# Autodesk Inventor assembly: structure_front
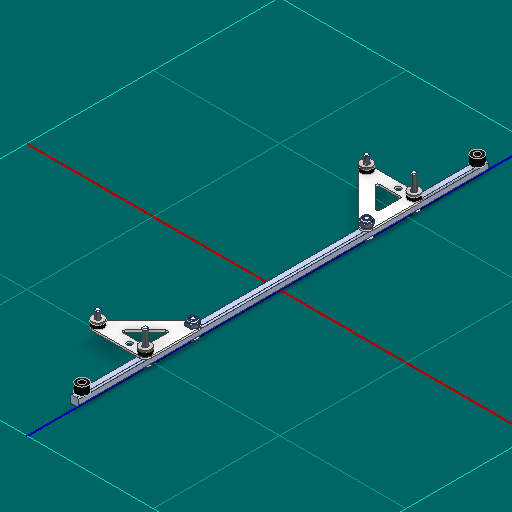
[picture p0: Inventor's stored thumbnail of the model, 512x512]
Saved by Autodesk Inventor 2025 (Build 290162000, 162)
## iProperties
Created: 2024-08-21
Part Number: structure_front
Document SubType Name: Assembly
Designer: averey
Author: averey
## Documents named in this file (12)
- C:\Users\avere\vex_robotics_high_stakes\hardware\cad\bots\ENIGMA\chassis\drivetrain\structure\structure_front.iam
- C:\Users\avere\vex_robotics_high_stakes\hardware\cad\bots\ENIGMA\chassis\drivetrain\structure\custom_parts\hs_crossbrace.ipt
- C:\Users\avere\vex_robotics_high_stakes\hardware\cad\bots\ENIGMA\chassis\drivetrain\structure\custom_parts\right_angle_gusset.ipt
- C:\Users\avere\vex_robotics_high_stakes\hardware\cad\VEX-CAD-Inventor\Structure\Hardware\Screw Steel - Star.ipt
- C:\Users\avere\vex_robotics_high_stakes\hardware\cad\VEX-CAD-Inventor\Motion\Spacers\Spacer Nylon .375 OD\NSpacer .375 OD x .125.ipt
- C:\Users\avere\vex_robotics_high_stakes\hardware\cad\VEX-CAD-Inventor\Motion\Spacers\Spacer Nylon .375 OD.ipt
- C:\Users\avere\vex_robotics_high_stakes\hardware\cad\VEX-CAD-Inventor\Motion\Spacers\Washer Steel\SWasher .375 OD x .062500.ipt
- C:\Users\avere\vex_robotics_high_stakes\hardware\cad\VEX-CAD-Inventor\Motion\Spacers\Washer Steel.ipt
- C:\Users\avere\vex_robotics_high_stakes\hardware\cad\VEX-CAD-Inventor\Motion\Spacers\Spacer Nylon .375 OD\NSpacer .375 OD x .250.ipt
- C:\Users\avere\vex_robotics_high_stakes\hardware\cad\VEX-CAD-Inventor\Structure\Hardware\Screw Steel - Star\SScrew Star Smooth .500.ipt
- C:\Users\avere\vex_robotics_high_stakes\hardware\cad\VEX-CAD-Inventor\Structure\Hardware\Nut Thin Nylock.ipt
- C:\Users\avere\vex_robotics_high_stakes\hardware\cad\VEX-CAD-Inventor\Structure\Hardware\Screw Steel - Star\SScrew Star Smooth 1.000.ipt
## Components (21 placed, 8 different names)
1. hs_crossbrace:1 — Mate:1, Insert:1, Mate:2, Insert:2, Mate:3, Insert:15, Insert:16, Insert:23, Insert:24, Insert:27, Insert:28
2. right_angle_gusset:1 — Insert:1, Mate:2, Insert:14, Insert:18, Insert:21, Insert:26
3. right_angle_gusset:2 — Insert:2, Mate:3, Insert:10, Insert:20, Insert:22, Insert:25
4. NSpacer .375 OD x .125:3 — Insert:10
5. SWasher .375 OD x .062500:2
6. NSpacer .375 OD x .125:5 — Insert:14
7. SWasher .375 OD x .062500:4
8. NSpacer .375 OD x .250:6 — Insert:15
9. NSpacer .375 OD x .250:7 — Insert:16
10. NSpacer .375 OD x .125:8 — Insert:18
11. SWasher .375 OD x .062500:5
12. NSpacer .375 OD x .125:9 — Insert:20
13. SWasher .375 OD x .062500:6
14. SScrew Star Smooth .500:6 — Insert:21
15. SScrew Star Smooth .500:7 — Insert:22
16. SScrew Star Smooth .500:8 — Insert:23
17. SScrew Star Smooth .500:9 — Insert:24
18. Nut Thin Nylock:1 — Insert:25
19. Nut Thin Nylock:2 — Insert:26
20. SScrew Star Smooth 1.000:10 — Insert:27
21. SScrew Star Smooth 1.000:11 — Insert:28
## Relationships (23: Insert 20, Mate 3)
- Mate:1 (-165.1 mm): hs_crossbrace:1
- Insert:1: hs_crossbrace:1 ↔ right_angle_gusset:1
- Mate:2: hs_crossbrace:1 ↔ right_angle_gusset:1
- Insert:2: hs_crossbrace:1 ↔ right_angle_gusset:2
- Mate:3: hs_crossbrace:1 ↔ right_angle_gusset:2
- [Insert]: NSpacer .375 OD x .125:3 ↔ SWasher .375 OD x .062500:2
- Insert:10: right_angle_gusset:2 ↔ NSpacer .375 OD x .125:3
- [Insert]: NSpacer .375 OD x .125:5 ↔ SWasher .375 OD x .062500:4
- Insert:14: right_angle_gusset:1 ↔ NSpacer .375 OD x .125:5
- Insert:15: hs_crossbrace:1 ↔ NSpacer .375 OD x .250:6
- Insert:16: hs_crossbrace:1 ↔ NSpacer .375 OD x .250:7
- [Insert]: NSpacer .375 OD x .125:8 ↔ SWasher .375 OD x .062500:5
- Insert:18: right_angle_gusset:1 ↔ NSpacer .375 OD x .125:8
- [Insert]: NSpacer .375 OD x .125:9 ↔ SWasher .375 OD x .062500:6
- Insert:20: right_angle_gusset:2 ↔ NSpacer .375 OD x .125:9
- Insert:21: right_angle_gusset:1 ↔ SScrew Star Smooth .500:6
- Insert:22: right_angle_gusset:2 ↔ SScrew Star Smooth .500:7
- Insert:23: hs_crossbrace:1 ↔ SScrew Star Smooth .500:8
- Insert:24: hs_crossbrace:1 ↔ SScrew Star Smooth .500:9
- Insert:25: right_angle_gusset:2 ↔ Nut Thin Nylock:1
- Insert:26: right_angle_gusset:1 ↔ Nut Thin Nylock:2
- Insert:27: hs_crossbrace:1 ↔ SScrew Star Smooth 1.000:10
- Insert:28: hs_crossbrace:1 ↔ SScrew Star Smooth 1.000:11
## Named parameters: d11_d9 = 0 mm, d14_d9 = 0 mm, d19_d14_d9 = 0 mm, d21_d14_d9 = 0 mm
